# Autodesk Inventor assembly: V4SlapperTower2
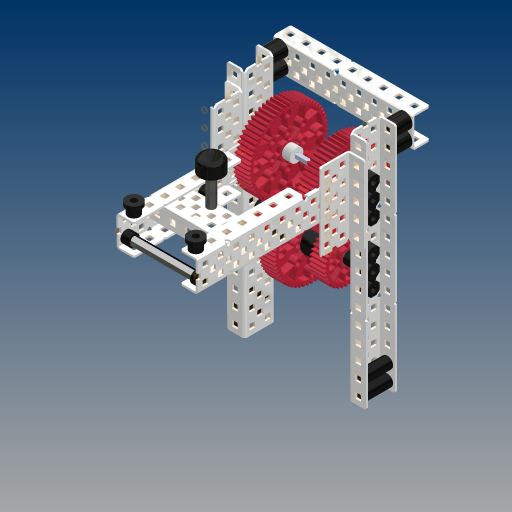
[picture p0: Inventor's stored thumbnail of the model, 512x512]
Saved by Autodesk Inventor 2023 (Build 270158000, 158)
## iProperties
Created: 2024-02-01
Part Number: V4SlapperTower2
Document SubType Name: Assembly
Designer: eddie
Author: eddie
## Documents named in this file (25)
- C:\Users\eddie\Documents\81208X-Over-Under-CAD\V4\V4SlapperTower2.iam
- C:\Users\eddie\Documents\81208X-Over-Under-CAD\VEX-CAD-Inventor-1.4.0\Structure\C Channel\Aluminum 1x2x1\Alu C 1x2x1x15.ipt
- C:\Users\eddie\Documents\81208X-Over-Under-CAD\Custom-parts\2x5 channel without 1 side.ipt
- C:\Users\eddie\Documents\81208X-Over-Under-CAD\VEX-CAD-Inventor-1.4.0\Motion\Shaft LS\Bearing Flat.ipt
- C:\Users\eddie\Documents\81208X-Over-Under-CAD\VEX-CAD-Inventor-1.4.0\Motion\Spacers\Spacer Nylon .375 OD\NSpacer .375 OD x .500.ipt
- C:\Users\eddie\Documents\81208X-Over-Under-CAD\VEX-CAD-Inventor-1.4.0\Motion\Spacers\Spacer Nylon .375 OD.ipt
- C:\Users\eddie\Documents\81208X-Over-Under-CAD\VEX-CAD-Inventor-1.4.0\Motion\Spacers\Spacer Nylon .375 OD\NSpacer .375 OD x .375.ipt
- C:\Users\eddie\Documents\81208X-Over-Under-CAD\Custom-parts\2x12 channel with 5 holes cut.ipt
- C:\Users\eddie\Documents\81208X-Over-Under-CAD\VEX-CAD-Inventor-1.4.0\Motion\Gears\HS Gear\HS 60T Gear, Square.iam
- C:\Users\eddie\Documents\81208X-Over-Under-CAD\VEX-CAD-Inventor-1.4.0\Motion\Gears\HS Gear.iam
- C:\Users\eddie\Documents\81208X-Over-Under-CAD\Custom-parts\Shaft Collar.ipt
- C:\Users\eddie\Documents\81208X-Over-Under-CAD\VEX-CAD-Inventor-1.4.0\Motion\Gears\HS Gear\HS 36T Gear, Square.iam
- C:\Users\eddie\Documents\81208X-Over-Under-CAD\VEX-CAD-Inventor-1.4.0\Motion\Spacers\Spacer Nylon .375 OD\NSpacer .375 OD x .250.ipt
- C:\Users\eddie\Documents\81208X-Over-Under-CAD\VEX-CAD-Inventor-1.4.0\Motion\Shaft HS\HS Shaft Collar.ipt
- C:\Users\eddie\Documents\81208X-Over-Under-CAD\VEX-CAD-Inventor-1.4.0\Structure\Standoff\Standoff 2.00.ipt
- C:\Users\eddie\Documents\81208X-Over-Under-CAD\VEX-CAD-Inventor-1.4.0\Structure\Standoff.ipt
- C:\Users\eddie\Documents\81208X-Over-Under-CAD\VEX-CAD-Inventor-1.4.0\Motion\Shaft LS\Shaft LS\Shaft LS 1.5.ipt
- C:\Users\eddie\Documents\81208X-Over-Under-CAD\VEX-CAD-Inventor-1.4.0\Motion\Shaft LS\Shaft LS.ipt
- C:\Users\eddie\Documents\81208X-Over-Under-CAD\VEX-CAD-Inventor-1.4.0\Structure\C Channel\Aluminum 1x2x1\Alu C 1x2x1x5.ipt
- C:\Users\eddie\Documents\81208X-Over-Under-CAD\VEX-CAD-Inventor-1.4.0\Structure\Hardware\Rubber Bumper Smooth.ipt
- C:\Users\eddie\Documents\81208X-Over-Under-CAD\VEX-CAD-Inventor-1.4.0\Structure\Standoff\Standoff 1.00.ipt
- C:\Users\eddie\Documents\81208X-Over-Under-CAD\VEX-CAD-Inventor-1.4.0\Motion\Spacers\Spacer Nylon .500 OD\NSpacer Black .500 OD x .125.ipt
- C:\Users\eddie\Documents\81208X-Over-Under-CAD\VEX-CAD-Inventor-1.4.0\Motion\Spacers\Spacer Nylon .500 OD.ipt
- C:\Users\eddie\Documents\81208X-Over-Under-CAD\VEX-CAD-Inventor-1.4.0\Motion\Spacers\Spacer Nylon .500 OD\NSpacer Black .500 OD x .500.ipt
- C:\Users\eddie\Documents\81208X-Over-Under-CAD\VEX-CAD-Inventor-1.4.0\Structure\C Channel\Aluminum 1x2x1\Alu C 1x2x1x9.ipt
## Components (50 placed, 19 different names)
1. Alu C 1x2x1x15:1 — Insert:2, Insert:5, Insert:6, Insert:11, Insert:12, Insert:15, Insert:24, Insert:49, Insert:50
2. Alu C 1x2x1x15:2 — Insert:1, Insert:3, Insert:4, Insert:7, Insert:8, Insert:16, Insert:23, Insert:47, Insert:48
3. 2x5 channel without 1 side:1 — Insert:2
4. 2x5 channel without 1 side:2 — Insert:1
5. Bearing Flat:1 — Insert:3
6. Bearing Flat:2 — Insert:4
7. Bearing Flat:3 — Insert:5
8. Bearing Flat:4 — Insert:6
9. NSpacer .375 OD x .500:1 — Insert:8, Insert:9
10. NSpacer .375 OD x .500:2 — Insert:7, Insert:10
11. NSpacer .375 OD x .375:3 — Insert:10
12. NSpacer .375 OD x .375:4 — Insert:9
13. NSpacer .375 OD x .500:5 — Insert:12, Insert:13
14. NSpacer .375 OD x .500:6 — Insert:11, Insert:14
15. NSpacer .375 OD x .375:7 — Insert:13
16. NSpacer .375 OD x .375:8 — Insert:14
17. NSpacer .375 OD x .375:9 — Insert:15, Insert:17
18. NSpacer .375 OD x .375:10 — Insert:16, Insert:18
19. 2x12 channel with 5 holes cut:1 — Insert:18, Insert:19, Insert:34, Insert:38, Insert:40, Insert:43
20. 2x12 channel with 5 holes cut:2 — Insert:17, Insert:20, Insert:33, Insert:39, Insert:44
21. HS 60T Gear, Square:1 [sub-assembly] — Insert:20, Insert:21
22. HS 60T Gear, Square:2 [sub-assembly] — Insert:19, Insert:22
23. Shaft Collar:1 — Insert:21, Insert:37
24. Shaft Collar:2 — Insert:22
25. NSpacer .375 OD x .500:11 — Insert:23, Insert:26
26. NSpacer .375 OD x .500:12 — Insert:24, Insert:25
27. HS 36T Gear, Square:3 [sub-assembly] — Insert:26, Insert:30
28. HS 36T Gear, Square:4 [sub-assembly] — Insert:25, Insert:27
29. NSpacer .375 OD x .250:13 — Insert:27, Insert:28
30. HS 60T Gear, Square:5 [sub-assembly] — Insert:28, Insert:29
31. HS Shaft Collar:1 — Insert:29
32. NSpacer .375 OD x .250:14 — Insert:30
33. NSpacer .375 OD x .250:15 — Insert:33, Insert:35
34. NSpacer .375 OD x .250:16 — Insert:34, Insert:36
35. Standoff 2.00:1 — Insert:35, Insert:36
36. Shaft LS 1.5:1 — Insert:37
37. Alu C 1x2x1x5:1 — Insert:38, Insert:41
38. NSpacer .375 OD x .250:17 — Insert:39
39. NSpacer .375 OD x .250:18 — Insert:40
40. Rubber Bumper Smooth:1 — Insert:42
41. Standoff 1.00:2 — Insert:41, Insert:42
42. NSpacer .375 OD x .250:19 — Insert:44, Insert:46
43. NSpacer .375 OD x .250:20 — Insert:43, Insert:45
44. NSpacer Black .500 OD x .125:1 — Insert:45
45. NSpacer Black .500 OD x .125:2 — Insert:46
46. NSpacer Black .500 OD x .500:3 — Insert:49
47. NSpacer Black .500 OD x .500:4 — Insert:50
48. NSpacer Black .500 OD x .500:5 — Insert:47, Insert:51
49. NSpacer Black .500 OD x .500:6 — Insert:48
50. Alu C 1x2x1x9:1 — Insert:51
## Relationships (49: Insert 49)
- Insert:1: Alu C 1x2x1x15:2 ↔ 2x5 channel without 1 side:2
- Insert:2: Alu C 1x2x1x15:1 ↔ 2x5 channel without 1 side:1
- Insert:3: Alu C 1x2x1x15:2 ↔ Bearing Flat:1
- Insert:4: Alu C 1x2x1x15:2 ↔ Bearing Flat:2
- Insert:5: Alu C 1x2x1x15:1 ↔ Bearing Flat:3
- Insert:6: Alu C 1x2x1x15:1 ↔ Bearing Flat:4
- Insert:7: Alu C 1x2x1x15:2 ↔ NSpacer .375 OD x .500:2
- Insert:8: Alu C 1x2x1x15:2 ↔ NSpacer .375 OD x .500:1
- Insert:9: NSpacer .375 OD x .500:1 ↔ NSpacer .375 OD x .375:4
- Insert:10: NSpacer .375 OD x .500:2 ↔ NSpacer .375 OD x .375:3
- Insert:11: Alu C 1x2x1x15:1 ↔ NSpacer .375 OD x .500:6
- Insert:12: Alu C 1x2x1x15:1 ↔ NSpacer .375 OD x .500:5
- Insert:13: NSpacer .375 OD x .500:5 ↔ NSpacer .375 OD x .375:7
- Insert:14: NSpacer .375 OD x .500:6 ↔ NSpacer .375 OD x .375:8
- Insert:15: Alu C 1x2x1x15:1 ↔ NSpacer .375 OD x .375:9
- Insert:16: Alu C 1x2x1x15:2 ↔ NSpacer .375 OD x .375:10
- Insert:17: NSpacer .375 OD x .375:9 ↔ 2x12 channel with 5 holes cut:2
- Insert:18: NSpacer .375 OD x .375:10 ↔ 2x12 channel with 5 holes cut:1
- Insert:19: 2x12 channel with 5 holes cut:1 ↔ HS 60T Gear, Square:2
- Insert:20: 2x12 channel with 5 holes cut:2 ↔ HS 60T Gear, Square:1
- Insert:21: HS 60T Gear, Square:1 ↔ Shaft Collar:1
- Insert:22: HS 60T Gear, Square:2 ↔ Shaft Collar:2
- Insert:23: Alu C 1x2x1x15:2 ↔ NSpacer .375 OD x .500:11
- Insert:24: Alu C 1x2x1x15:1 ↔ NSpacer .375 OD x .500:12
- Insert:25: NSpacer .375 OD x .500:12 ↔ HS 36T Gear, Square:4
- Insert:26: NSpacer .375 OD x .500:11 ↔ HS 36T Gear, Square:3
- Insert:27: HS 36T Gear, Square:4 ↔ NSpacer .375 OD x .250:13
- Insert:28: NSpacer .375 OD x .250:13 ↔ HS 60T Gear, Square:5
- Insert:29: HS 60T Gear, Square:5 ↔ HS Shaft Collar:1
- Insert:30: HS 36T Gear, Square:3 ↔ NSpacer .375 OD x .250:14
- Insert:33: 2x12 channel with 5 holes cut:2 ↔ NSpacer .375 OD x .250:15
- Insert:34: 2x12 channel with 5 holes cut:1 ↔ NSpacer .375 OD x .250:16
- Insert:35: NSpacer .375 OD x .250:15 ↔ Standoff 2.00:1
- Insert:36: NSpacer .375 OD x .250:16 ↔ Standoff 2.00:1
- Insert:37: Shaft Collar:1 ↔ Shaft LS 1.5:1
- Insert:38: 2x12 channel with 5 holes cut:1 ↔ Alu C 1x2x1x5:1
- Insert:39: 2x12 channel with 5 holes cut:2 ↔ NSpacer .375 OD x .250:17
- Insert:40: 2x12 channel with 5 holes cut:1 ↔ NSpacer .375 OD x .250:18
- Insert:41: Alu C 1x2x1x5:1 ↔ Standoff 1.00:2
- Insert:42: Rubber Bumper Smooth:1 ↔ Standoff 1.00:2
- Insert:43: 2x12 channel with 5 holes cut:1 ↔ NSpacer .375 OD x .250:20
- Insert:44: 2x12 channel with 5 holes cut:2 ↔ NSpacer .375 OD x .250:19
- Insert:45: NSpacer .375 OD x .250:20 ↔ NSpacer Black .500 OD x .125:1
- Insert:46: NSpacer .375 OD x .250:19 ↔ NSpacer Black .500 OD x .125:2
- Insert:47: Alu C 1x2x1x15:2 ↔ NSpacer Black .500 OD x .500:5
- Insert:48: Alu C 1x2x1x15:2 ↔ NSpacer Black .500 OD x .500:6
- Insert:49: Alu C 1x2x1x15:1 ↔ NSpacer Black .500 OD x .500:3
- Insert:50: Alu C 1x2x1x15:1 ↔ NSpacer Black .500 OD x .500:4
- Insert:51: NSpacer Black .500 OD x .500:5 ↔ Alu C 1x2x1x9:1
